# Autodesk Inventor assembly: LearningKitSolarAlt
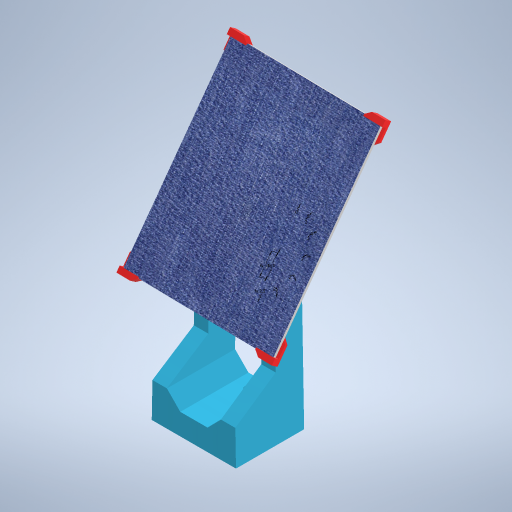
[picture p0: Inventor's stored thumbnail of the model, 512x512]
Saved by Autodesk Inventor 2024.3 (Build 283343000, 343)
## iProperties
Created: 2025-02-03
Part Number: LearningKitSolarAlt
Document SubType Name: Assembly
Designer: Maximilian Hock
Author: Maximilian Hock
## Documents named in this file (6)
- Z:\Dokumente\LearningKit\LearningKitSolar\LearningKitSolar.iam
- Z:\Dokumente\LearningKit\LearningKitSolar\SolarCradle.ipt
- Z:\Dokumente\LearningKit\LearningKitSolar\SolarFoot.ipt
- Z:\Dokumente\LearningKit\LearningKitSolar\SolarScale.ipt
- Z:\Dokumente\LearningKit\LearningKitSolar\SolarPanel.ipt
- Z:\Dokumente\LearningKit\LearningKitSolar\SolarPlugAdapter.ipt
## Components (6 placed, 5 different names)
1. SolarCradle:1 — Starr:2, Starr:3
2. SolarFoot:1 — Passend:1, Passend:3, Passend:4, Einfügen:1
3. SolarScale:1 — Starr:3, Einfügen:1
4. SolarPanel:1 — Starr:2
5. SolarPlugAdapter:1
6. SolarPlugAdapter:2
## Relationships (6: Mate 3, WeldJoint 2, Insert 1)
- Passend:1 [Mate]: SolarFoot:1
- Passend:3 [Mate]: SolarFoot:1
- Starr:2 [WeldJoint]: SolarCradle:1 ↔ SolarPanel:1
- Passend:4 [Mate]: SolarFoot:1
- Starr:3 [WeldJoint]: SolarCradle:1 ↔ SolarScale:1
- Einfügen:1 [Insert]: SolarFoot:1 ↔ SolarScale:1
